# Autodesk Inventor assembly: small-model-rocket-launch-pad
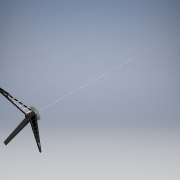
[picture p0: Inventor's stored thumbnail of the model, 180x180]
Saved by Autodesk Inventor 2017 (Build 210142000, 142)
## iProperties
Created: 2020-06-17
Part Number: small-model-rocket-launch-pad
Document SubType Name: Assembly
Designer: HAYNIE R&D
Mass: 395.282 g
Surface Area: 1499.44 cm^2
Volume: 372.908 cm^3
Density: 1.06 g/cm^3
Author: HAYNIE R&D
## Documents named in this file (11)
- C:\Users\HAYNIE\source\repos\small-model-rocket-launch-pad\small-model-rocket-launch-pad.iam
- C:\Users\HAYNIE\source\repos\small-model-rocket-launch-pad\center.ipt
- C:\Users\HAYNIE\source\repos\small-model-rocket-launch-pad\leg.ipt
- C:\Users\HAYNIE\source\repos\small-model-rocket-launch-pad\rod.ipt
- C:\Users\HAYNIE\source\repos\small-model-rocket-launch-pad\plate.ipt
- C:\Users\HAYNIE\source\repos\small-model-rocket-launch-pad\small-model-rocket-launch-pad\AIP\FEA\d9x4y7qsg.fins
- C:\Users\HAYNIE\source\repos\small-model-rocket-launch-pad\small-model-rocket-launch-pad\AIP\FEA\d9x4y7qsg.fsat
- C:\Users\HAYNIE\source\repos\small-model-rocket-launch-pad\small-model-rocket-launch-pad\AIP\FEA\d9x4y7qsg.ftes
- C:\Users\HAYNIE\source\repos\small-model-rocket-launch-pad\small-model-rocket-launch-pad\AIP\FEA\d9x4y7qsg.fwiz
- C:\Users\HAYNIE\source\repos\small-model-rocket-launch-pad\small-model-rocket-launch-pad\AIP\FEA\d9x4y7qu8.fmsh
- C:\Users\HAYNIE\source\repos\small-model-rocket-launch-pad\small-model-rocket-launch-pad\AIP\FEA\d9x4y7qu9.fres
## Components (6 placed, 4 different names)
1. center:1 — Slider:2, Slider:4, Slider:5, Rigid:1, Rotational:1
2. leg:1 — Slider:2
3. leg:2 — Slider:5
4. leg:3 — Slider:4
5. rod:1 — Rigid:1
6. plate:1 — Rotational:1
## Relationships (5: TranslationJoint 3, WeldJoint 1, RevoluteJoint 1)
- Slider:2 [TranslationJoint]: center:1 ↔ leg:1
- Slider:4 [TranslationJoint]: center:1 ↔ leg:3
- Slider:5 [TranslationJoint]: center:1 ↔ leg:2
- Rigid:1 [WeldJoint]: center:1 ↔ rod:1
- Rotational:1 [RevoluteJoint] (-1 mm): center:1 ↔ plate:1
## Named parameters: sa_0 = 45000
note: some values were not read from the file. Shown as the stored number, unit unknown: "sa_0".
